# Autodesk Inventor assembly: Base Plate Assembly
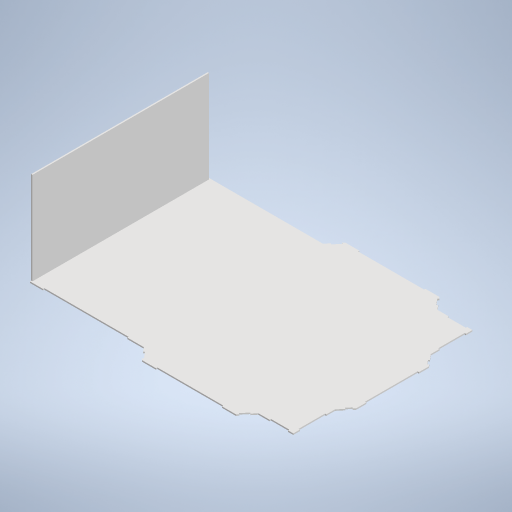
[picture p0: Inventor's stored thumbnail of the model, 512x512]
Saved by Autodesk Inventor 2023 (Build 270158000, 158)
## iProperties
Created: 2023-02-07
Part Number: Base Plate Assembly
Document SubType Name: Assembly
Designer: cheng
Author: cheng
## Documents named in this file (3)
- C:\Users\cheng\Desktop\4th Year Project\Inventor\12th Assembly\Base Plate V2\Base Plate Assembly.iam
- C:\Users\cheng\Desktop\4th Year Project\Inventor\12th Assembly\Base Plate V2\Base Plate.ipt
- C:\Users\cheng\Desktop\4th Year Project\Inventor\12th Assembly\Base Plate V2\Base Plate Wall 1.ipt
## Components (2 placed, 2 different names)
1. Base Plate:1 — Mate:1, Flush:1, Mate:2
2. Base Plate Wall 1:1 — Mate:1, Flush:1, Mate:2
## Relationships (3: Mate 2, Flush 1)
- Mate:1: Base Plate:1 ↔ Base Plate Wall 1:1
- Flush:1: Base Plate:1 ↔ Base Plate Wall 1:1
- Mate:2: Base Plate:1 ↔ Base Plate Wall 1:1
